# Autodesk Inventor assembly: B_Legs0
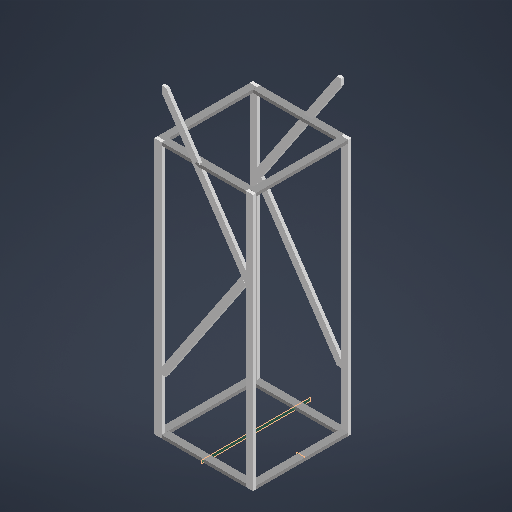
[picture p0: Inventor's stored thumbnail of the model, 512x512]
Saved by Autodesk Inventor 2026 (Build 300175000, 175)
## iProperties
Created: 2024-09-19
Part Number: B_Legs0
Document SubType Name: Assembly
Designer: User
Author: User
## Documents named in this file (6)
- C:\Users\trott\Documents\UofSC-ASME-Tiger-Burn-Design-2025\CAD\Legs\Front Leg\F_Leg.iam
- C:\Users\trott\Documents\UofSC-ASME-Tiger-Burn-Design-2025\CAD\Legs\Front Leg\2x4x42.ipt
- C:\Users\trott\Documents\UofSC-ASME-Tiger-Burn-Design-2025\CAD\Legs\Front Leg\2x4x125.ipt
- C:\Users\trott\Documents\UofSC-ASME-Tiger-Burn-Design-2025\CAD\Legs\Front Leg\S_2x4x76.102.ipt
- C:\Users\trott\Documents\UofSC-ASME-Tiger-Burn-Design-2025\CAD\Legs\Front Leg\S_2x4x95.725.ipt
- C:\Users\trott\Documents\UofSC-ASME-Tiger-Burn-Design-2025\CAD\Legs\Front Leg\2x4x45.ipt
## Components (16 placed, 5 different names)
1. 2x4x42:5 — Flush:27, Mate:18, Flush:28, Mate:34
2. S_2x4x76.102:1 — Flush:45
3. S_2x4x76.102:2 — Mate:29, Flush:46
4. S_2x4x95.725:1 — Mate:31, Flush:47
5. S_2x4x95.725:2 — Mate:33, Mate:34, Flush:48
6. 2x4x45:1 — Mate:35, Flush:49, Mate:37, Mate:39, Flush:52
7. 2x4x42:6 — Mate:38, Flush:50, Flush:51, Mate:41
8. 2x4x42:7 — Mate:39, Flush:52, Flush:53
9. 2x4x45:2 — Mate:40, Flush:54, Mate:41
10. 2x4x45:3 — Mate:42, Flush:55, Flush:56
11. 2x4x45:4 — Mate:43, Flush:57, Flush:58, Flush:59, Flush:60
12. 2x4x42:8 — Mate:44, Flush:61, Flush:62
13. 2x4x125:2 — Mate:29, Flush:46, Mate:31, Flush:47, Mate:40, Flush:54, Mate:43, Flush:59, Flush:60
14. 2x4x125:1 — Flush:27, Mate:18, Flush:28, Flush:57, Flush:58
15. 2x4x125:3 — Mate:35, Flush:49, Mate:38, Flush:50, Flush:51, Mate:42, Mate:44, Flush:61, Flush:62
16. 2x4x125:4 — Flush:45, Mate:33, Flush:48, Mate:37, Flush:53, Flush:55, Flush:56
## Component patterns: (2 elements, first: 2x4x125:2 + 2x4x125:1)
## Relationships (34: Flush 20, Mate 14)
- Flush:27: 2x4x42:5 ↔ 2x4x125:1
- Mate:18: 2x4x42:5 ↔ 2x4x125:1
- Flush:28: 2x4x42:5 ↔ 2x4x125:1
- Flush:45: S_2x4x76.102:1 ↔ 2x4x125:4
- Mate:29: S_2x4x76.102:2 ↔ 2x4x125:2
- Flush:46: S_2x4x76.102:2 ↔ 2x4x125:2
- Mate:31: S_2x4x95.725:1 ↔ 2x4x125:2
- Flush:47: S_2x4x95.725:1 ↔ 2x4x125:2
- Mate:33: S_2x4x95.725:2 ↔ 2x4x125:4
- Mate:34: 2x4x42:5 ↔ S_2x4x95.725:2
- Flush:48: S_2x4x95.725:2 ↔ 2x4x125:4
- Mate:35: 2x4x45:1 ↔ 2x4x125:3
- Flush:49: 2x4x45:1 ↔ 2x4x125:3
- Mate:37: 2x4x45:1 ↔ 2x4x125:4
- Mate:38: 2x4x42:6 ↔ 2x4x125:3
- Flush:50: 2x4x42:6 ↔ 2x4x125:3
- Flush:51: 2x4x42:6 ↔ 2x4x125:3
- Mate:39: 2x4x45:1 ↔ 2x4x42:7
- Flush:52: 2x4x45:1 ↔ 2x4x42:7
- Flush:53: 2x4x42:7 ↔ 2x4x125:4
- Mate:40: 2x4x45:2 ↔ 2x4x125:2
- Flush:54: 2x4x45:2 ↔ 2x4x125:2
- Mate:41: 2x4x42:6 ↔ 2x4x45:2
- Mate:42: 2x4x45:3 ↔ 2x4x125:3
- Flush:55: 2x4x45:3 ↔ 2x4x125:4
- Flush:56: 2x4x45:3 ↔ 2x4x125:4
- Mate:43: 2x4x45:4 ↔ 2x4x125:2
- Flush:57: 2x4x45:4 ↔ 2x4x125:1
- Flush:58: 2x4x45:4 ↔ 2x4x125:1
- Flush:59: 2x4x45:4 ↔ 2x4x125:2
- Flush:60: 2x4x45:4 ↔ 2x4x125:2
- Mate:44: 2x4x42:8 ↔ 2x4x125:3
- Flush:61: 2x4x42:8 ↔ 2x4x125:3
- Flush:62: 2x4x42:8 ↔ 2x4x125:3
